# Autodesk Inventor assembly: Idler Assembly
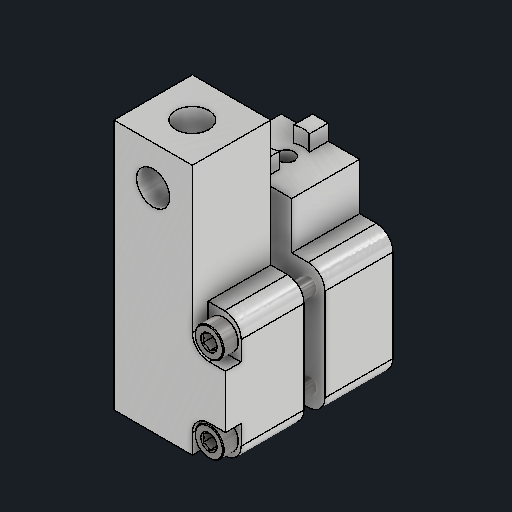
[picture p0: Inventor's stored thumbnail of the model, 512x512]
Saved by Autodesk Inventor 2026.2 (Build 302298000, 298)
## iProperties
Created: 2025-05-27
Part Number: Idler Assembly
Document SubType Name: Assembly
Designer: Joshua Eah
Author: Joshua Eah
## Documents named in this file (6)
- C:\Users\JoshuaEah\Documents\GitHub\Voron-0\CAD\Idlers\B Idler Assembly (Alternate).iam
- C:\Users\JoshuaEah\Documents\GitHub\Voron-0\CAD\Hardware\Bearings\F623 Stack.iam
- C:\Users\JoshuaEah\Documents\GitHub\Voron-0\CAD\Hardware\Fasteners\M3x20 SHCS.ipt
- C:\Users\JoshuaEah\Documents\GitHub\Voron-0\CAD\Idlers\Bearing Carriage.ipt
- C:\Users\JoshuaEah\Documents\GitHub\Voron-0\CAD\Idlers\B Idler (Alternate).ipt
- C:\Users\JoshuaEah\Documents\GitHub\Voron-0\CAD\Hardware\Pins\3x30 Pin.ipt
## Components (6 placed, 5 different names)
1. Bearing Carriage:1 — Mate:1, Mate:2, Insert:1, Insert:2, Mate:3
2. B Idler (Alternate):1 — Mate:1, Mate:2, Mate:3, Insert:3, Insert:4
3. F623 Stack:1 [sub-assembly] — Insert:1
4. 3x30 Pin:1 — Insert:2
5. M3x20 SHCS:1 — Insert:3
6. M3x20 SHCS:2 — Insert:4
## Relationships (7: Insert 4, Mate 3)
- Mate:1: Bearing Carriage:1 ↔ B Idler (Alternate):1
- Mate:2: Bearing Carriage:1 ↔ B Idler (Alternate):1
- Insert:1: Bearing Carriage:1 ↔ F623 Stack:1
- Insert:2: Bearing Carriage:1 ↔ 3x30 Pin:1
- Mate:3 (4 mm): Bearing Carriage:1 ↔ B Idler (Alternate):1
- Insert:3: B Idler (Alternate):1 ↔ M3x20 SHCS:1
- Insert:4: B Idler (Alternate):1 ↔ M3x20 SHCS:2
